# Autodesk Inventor assembly: SidePanel-noFibre
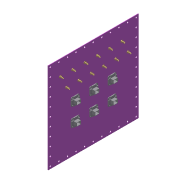
[picture p0: Inventor's stored thumbnail of the model, 180x180]
Saved by Autodesk Inventor 2017 (Build 210142000, 142)
## iProperties
Created: 2017-11-15
Part Number: SidePanel-noFibre
Document SubType Name: Assembly
Designer: Kathryn Rosie
Author: Kathryn Rosie
## Documents named in this file (4)
- C:\Users\Kathryn Rosie\Google Drive\HERA\hera-cad-0\Node\20171017 Node\SidePanel-noFibre.iam
- C:\Users\Kathryn Rosie\Google Drive\HERA\hera-cad-0\Node\20171017 Node\RD-A001-P001-REV0-noCutouts.ipt
- C:\Users\Kathryn Rosie\Google Drive\HERA\hera-cad-0\Node\20171017 Node\Interfaces\SMA_bulkhead\132170_3d_model_file.iam
- C:\Users\Kathryn Rosie\Google Drive\HERA\hera-cad-0\Node\20171017 Node\RJ45Assy.iam
## Components (19 placed, 3 different names)
1. RD-A001-P001-REV0-noCutouts:1 — Mate:1, Mate:2, Mate:3, Mate:4, Mate:5, Mate:6, Mate:7, Mate:8, Mate:9, Mate:10, Mate:11, Mate:12, Angle:1, Angle:2, Angle:3, Angle:4, Angle:5, Angle:6, Angle:7, Angle:8, Angle:9, Angle:10, Angle:11, Angle:12, Mate:13, Mate:14, Mate:15, Mate:16, Mate:17, Mate:18, Mate:19, Mate:20, Mate:21, Mate:22, Mate:23, Mate:24, Mate:25, Mate:26, Mate:27, Mate:28, Mate:29, Mate:30, Mate:31, Mate:32, Mate:33, Mate:34, Mate:35, Mate:36, Mate:37, Mate:38, Mate:39, Mate:40, Mate:41, Mate:42
2. 132170_3d_model_file:1 [sub-assembly] — Mate:11, Angle:11, Mate:15
3. 132170_3d_model_file:2 [sub-assembly] — Mate:9, Angle:9, Mate:17
4. 132170_3d_model_file:3 [sub-assembly] — Mate:7, Angle:7, Mate:19
5. 132170_3d_model_file:4 [sub-assembly] — Mate:5, Angle:5, Mate:21
6. 132170_3d_model_file:5 [sub-assembly] — Mate:4, Angle:4, Mate:20
7. 132170_3d_model_file:6 [sub-assembly] — Mate:2, Angle:1, Mate:24
8. 132170_3d_model_file:7 [sub-assembly] — Mate:12, Angle:12, Mate:13
9. 132170_3d_model_file:8 [sub-assembly] — Mate:10, Angle:10, Mate:14
10. 132170_3d_model_file:9 [sub-assembly] — Mate:8, Angle:8, Mate:16
11. 132170_3d_model_file:10 [sub-assembly] — Mate:6, Angle:6, Mate:18
12. 132170_3d_model_file:11 [sub-assembly] — Mate:3, Angle:3, Mate:23
13. 132170_3d_model_file:12 [sub-assembly] — Mate:1, Angle:2, Mate:22
14. RJ45Assy:1 [sub-assembly] — Mate:25, Mate:35, Mate:36
15. RJ45Assy:2 [sub-assembly] — Mate:26, Mate:33, Mate:34
16. RJ45Assy:3 [sub-assembly] — Mate:28, Mate:37, Mate:38
17. RJ45Assy:4 [sub-assembly] — Mate:29, Mate:39, Mate:40
18. RJ45Assy:5 [sub-assembly] — Mate:27, Mate:31, Mate:32
19. RJ45Assy:6 [sub-assembly] — Mate:30, Mate:41, Mate:42
## Relationships (54: Mate 42, Angle 12)
- Mate:1: RD-A001-P001-REV0-noCutouts:1 ↔ 132170_3d_model_file:12
- Mate:2: RD-A001-P001-REV0-noCutouts:1 ↔ 132170_3d_model_file:6
- Mate:3: RD-A001-P001-REV0-noCutouts:1 ↔ 132170_3d_model_file:11
- Mate:4: RD-A001-P001-REV0-noCutouts:1 ↔ 132170_3d_model_file:5
- Mate:5: RD-A001-P001-REV0-noCutouts:1 ↔ 132170_3d_model_file:4
- Mate:6: RD-A001-P001-REV0-noCutouts:1 ↔ 132170_3d_model_file:10
- Mate:7: RD-A001-P001-REV0-noCutouts:1 ↔ 132170_3d_model_file:3
- Mate:8: RD-A001-P001-REV0-noCutouts:1 ↔ 132170_3d_model_file:9
- Mate:9: RD-A001-P001-REV0-noCutouts:1 ↔ 132170_3d_model_file:2
- Mate:10: RD-A001-P001-REV0-noCutouts:1 ↔ 132170_3d_model_file:8
- Mate:11: RD-A001-P001-REV0-noCutouts:1 ↔ 132170_3d_model_file:1
- Mate:12: RD-A001-P001-REV0-noCutouts:1 ↔ 132170_3d_model_file:7
- Angle:1 (180 deg): RD-A001-P001-REV0-noCutouts:1 ↔ 132170_3d_model_file:6
- Angle:2 (180 deg): RD-A001-P001-REV0-noCutouts:1 ↔ 132170_3d_model_file:12
- Angle:3 (180 deg): RD-A001-P001-REV0-noCutouts:1 ↔ 132170_3d_model_file:11
- Angle:4 (180 deg): RD-A001-P001-REV0-noCutouts:1 ↔ 132170_3d_model_file:5
- Angle:5 (180 deg): RD-A001-P001-REV0-noCutouts:1 ↔ 132170_3d_model_file:4
- Angle:6 (180 deg): RD-A001-P001-REV0-noCutouts:1 ↔ 132170_3d_model_file:10
- Angle:7 (180 deg): RD-A001-P001-REV0-noCutouts:1 ↔ 132170_3d_model_file:3
- Angle:8 (180 deg): RD-A001-P001-REV0-noCutouts:1 ↔ 132170_3d_model_file:9
- Angle:9 (180 deg): RD-A001-P001-REV0-noCutouts:1 ↔ 132170_3d_model_file:2
- Angle:10 (180 deg): RD-A001-P001-REV0-noCutouts:1 ↔ 132170_3d_model_file:8
- Angle:11 (180 deg): RD-A001-P001-REV0-noCutouts:1 ↔ 132170_3d_model_file:1
- Angle:12 (180 deg): RD-A001-P001-REV0-noCutouts:1 ↔ 132170_3d_model_file:7
- Mate:13: RD-A001-P001-REV0-noCutouts:1 ↔ 132170_3d_model_file:7
- Mate:14: RD-A001-P001-REV0-noCutouts:1 ↔ 132170_3d_model_file:8
- Mate:15: RD-A001-P001-REV0-noCutouts:1 ↔ 132170_3d_model_file:1
- Mate:16: RD-A001-P001-REV0-noCutouts:1 ↔ 132170_3d_model_file:9
- Mate:17: RD-A001-P001-REV0-noCutouts:1 ↔ 132170_3d_model_file:2
- Mate:18: RD-A001-P001-REV0-noCutouts:1 ↔ 132170_3d_model_file:10
- Mate:19: RD-A001-P001-REV0-noCutouts:1 ↔ 132170_3d_model_file:3
- Mate:20: RD-A001-P001-REV0-noCutouts:1 ↔ 132170_3d_model_file:5
- Mate:21: RD-A001-P001-REV0-noCutouts:1 ↔ 132170_3d_model_file:4
- Mate:22: RD-A001-P001-REV0-noCutouts:1 ↔ 132170_3d_model_file:12
- Mate:23: RD-A001-P001-REV0-noCutouts:1 ↔ 132170_3d_model_file:11
- Mate:24: RD-A001-P001-REV0-noCutouts:1 ↔ 132170_3d_model_file:6
- Mate:25: RD-A001-P001-REV0-noCutouts:1 ↔ RJ45Assy:1
- Mate:26: RD-A001-P001-REV0-noCutouts:1 ↔ RJ45Assy:2
- Mate:27: RD-A001-P001-REV0-noCutouts:1 ↔ RJ45Assy:5
- Mate:28: RD-A001-P001-REV0-noCutouts:1 ↔ RJ45Assy:3
- Mate:29: RD-A001-P001-REV0-noCutouts:1 ↔ RJ45Assy:4
- Mate:30: RD-A001-P001-REV0-noCutouts:1 ↔ RJ45Assy:6
- Mate:31: RD-A001-P001-REV0-noCutouts:1 ↔ RJ45Assy:5
- Mate:32: RD-A001-P001-REV0-noCutouts:1 ↔ RJ45Assy:5
- Mate:33: RD-A001-P001-REV0-noCutouts:1 ↔ RJ45Assy:2
- Mate:34: RD-A001-P001-REV0-noCutouts:1 ↔ RJ45Assy:2
- Mate:35: RD-A001-P001-REV0-noCutouts:1 ↔ RJ45Assy:1
- Mate:36: RD-A001-P001-REV0-noCutouts:1 ↔ RJ45Assy:1
- Mate:37: RD-A001-P001-REV0-noCutouts:1 ↔ RJ45Assy:3
- Mate:38: RD-A001-P001-REV0-noCutouts:1 ↔ RJ45Assy:3
- Mate:39: RD-A001-P001-REV0-noCutouts:1 ↔ RJ45Assy:4
- Mate:40: RD-A001-P001-REV0-noCutouts:1 ↔ RJ45Assy:4
- Mate:41: RD-A001-P001-REV0-noCutouts:1 ↔ RJ45Assy:6
- Mate:42: RD-A001-P001-REV0-noCutouts:1 ↔ RJ45Assy:6
